# Autodesk Inventor assembly: Cierre Baño2
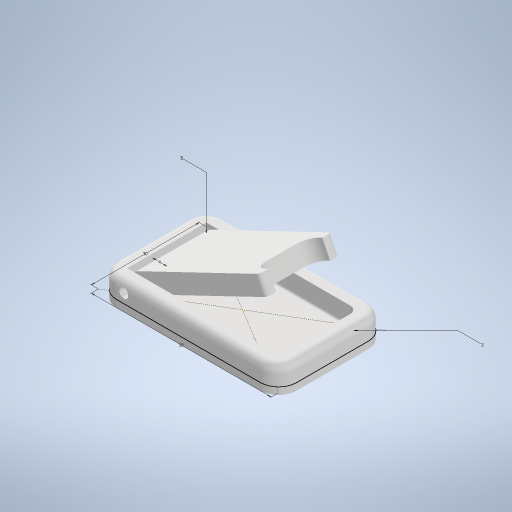
[picture p0: Inventor's stored thumbnail of the model, 512x512]
Saved by Autodesk Inventor 2024 (Build 280153000, 153)
## iProperties
Created: 2023-09-22
Part Number: Cierre Baño2
Document SubType Name: Assembly
Designer: sergi
Author: sergi
## Documents named in this file (3)
- C:\Users\sergi\OneDrive\Escritorio\Piso\Cierre Baño\Cierre Baño2.iam
- C:\Users\sergi\OneDrive\Escritorio\Piso\Cierre Baño\Base2.ipt
- C:\Users\sergi\OneDrive\Escritorio\Piso\Cierre Baño\Brazo2_2.ipt
## Components (2 placed, 2 different names)
1. Base2:1 — Coincidencia:1, Coincidencia:2
2. Brazo2_2:1 — Coincidencia:1, Coincidencia:2
## Relationships (2: Mate 2)
- Coincidencia:1 [Mate]: Base2:1 ↔ Brazo2_2:1
- Coincidencia:2 [Mate] (1 mm): Base2:1 ↔ Brazo2_2:1
